# Autodesk Inventor assembly: assy-box
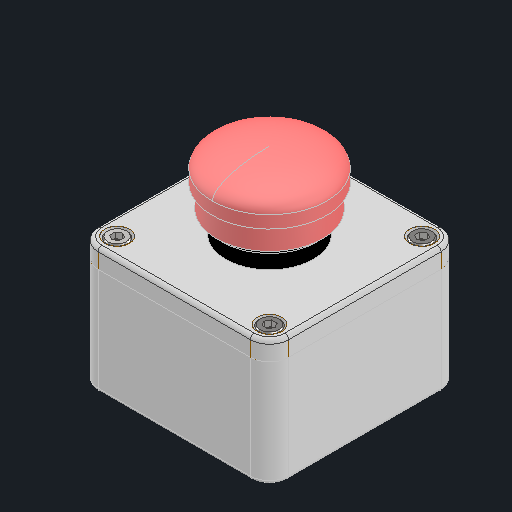
[picture p0: Inventor's stored thumbnail of the model, 512x512]
Saved by Autodesk Inventor 2022 (Build 260153000, 153)
## iProperties
Created: 2021-04-30
Part Number: assy-box
Document SubType Name: Assembly
Designer: yuta0
Author: yuta0
## Documents named in this file (9)
- C:\Users\yuta0\Documents\GitHub\catchrobo_hardware\emergency_switch_box\assy-box.iam
- C:\Users\yuta0\Documents\GitHub\catchrobo_hardware\emergency_switch_box\box.ipt
- C:\Users\yuta0\Documents\GitHub\catchrobo_hardware\emergency_switch_box\A165E_S_02.iam
- C:\Users\yuta0\Documents\GitHub\catchrobo_hardware\emergency_switch_box\box_top.ipt
- C:\Users\yuta0\Documents\GitHub\catchrobo_hardware\emergency_switch_box\box_bottom.ipt
- C:\Users\yuta0\Documents\GitHub\catchrobo_hardware\emergency_switch_box\LBNR3.ipt
- C:\Users\yuta0\Documents\GitHub\catchrobo_hardware\emergency_switch_box\CB3-30.ipt
- C:\Users\yuta0\Documents\GitHub\catchrobo_hardware\assy-robot\PLT-164-R-R.ipt
- C:\Users\yuta0\Documents\GitHub\catchrobo_hardware\assy-robot\holder_magnet.ipt
## Components (17 placed, 8 different names)
1. box:1 — メイト:1, 角度:1, メイト:2
2. A165E_S_02:1 [sub-assembly] — メイト:1, 角度:1, メイト:2
3. box_top:1 — メイト:6, メイト:7
4. box_bottom:1 — メイト:3, メイト:4, メイト:5, メイト:8, メイト:9, メイト:10, メイト:11, フラッシュ:1
5. PLT-164-R-R:1 — メイト:8, メイト:9, メイト:10
6. CB3-30:1 — メイト:6, メイト:7
7. LBNR3:1 — メイト:3, メイト:4, メイト:5
8. CB3-30:2
9. LBNR3:2
10. CB3-30:3
11. LBNR3:3
12. CB3-30:4
13. LBNR3:4
14. holder_magnet:1 — メイト:11, フラッシュ:1
15. holder_magnet:2
16. holder_magnet:3
17. holder_magnet:4
## Component patterns: (4 elements, first: CB3-30:1 + LBNR3:1), (4 elements, first: holder_magnet:1)
## Relationships (13: Mate 11, Angle 1, Flush 1)
- メイト:1 [Mate]: box:1 ↔ A165E_S_02:1
- 角度:1 [Angle] (0 deg): box:1 ↔ A165E_S_02:1
- メイト:2 [Mate]: box:1 ↔ A165E_S_02:1
- メイト:3 [Mate]: box_bottom:1 ↔ LBNR3:1
- メイト:4 [Mate]: box_bottom:1 ↔ LBNR3:1
- メイト:5 [Mate]: box_bottom:1 ↔ LBNR3:1
- メイト:6 [Mate]: box_top:1 ↔ CB3-30:1
- メイト:7 [Mate]: box_top:1 ↔ CB3-30:1
- メイト:8 [Mate]: box_bottom:1 ↔ PLT-164-R-R:1
- メイト:9 [Mate]: box_bottom:1 ↔ PLT-164-R-R:1
- メイト:10 [Mate]: box_bottom:1 ↔ PLT-164-R-R:1
- メイト:11 [Mate]: box_bottom:1 ↔ holder_magnet:1
- フラッシュ:1 [Flush]: box_bottom:1 ↔ holder_magnet:1
